# Autodesk Inventor assembly: PIVOT
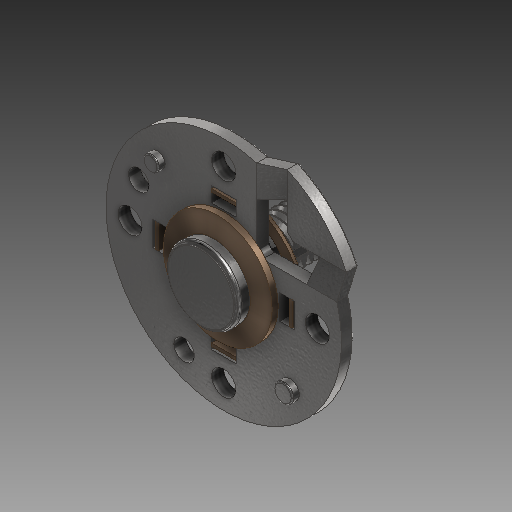
[picture p0: Inventor's stored thumbnail of the model, 512x512]
Saved by Autodesk Inventor 2017 SP1 (Build 210196100, 196)
## iProperties
Created: 2021-01-06
Part Number: PIVOT
Document SubType Name: Assembly
Designer: Napoleon
Author: Napoleon
## Documents named in this file (5)
- D:\PRYWATNE\PROJEKTY\POKÓJ\URZĄDZENIA PERYFERYJNE\DELL 1909Wf\BLOKADA.iam
- D:\PRYWATNE\PROJEKTY\POKÓJ\URZĄDZENIA PERYFERYJNE\DELL 1909Wf\ŚRUBA M8 Z WIĘCIAMI.ipt
- D:\PRYWATNE\PROJEKTY\POKÓJ\URZĄDZENIA PERYFERYJNE\DELL 1909Wf\PODKŁADKA SPRĘŻYNOWA M8X18.ipt
- D:\PRYWATNE\PROJEKTY\POKÓJ\URZĄDZENIA PERYFERYJNE\DELL 1909Wf\SŁONECZKO BLOKADY.ipt
- D:\PRYWATNE\PROJEKTY\POKÓJ\URZĄDZENIA PERYFERYJNE\DELL 1909Wf\BLOKADA PIVOT.ipt
## Components (4 placed, 4 different names)
1. ŚRUBA M8 Z WIĘCIAMI:1 — Obrotowe:1, Zestawiający:4, Zestawiający:5
2. PODKŁADKA SPRĘŻYNOWA M8X18:1 — Obrotowe:1, Zestawiający:6
3. BLOKADA PIVOT:1 — Zestawiający:4, Zestawiający:5, Zestawiający:6, Zestawiający:7
4. SŁONECZKO BLOKADY:1 — Zestawiający:7
## Relationships (5: Mate 4, RevoluteJoint 1)
- Obrotowe:1 [RevoluteJoint]: ŚRUBA M8 Z WIĘCIAMI:1 ↔ PODKŁADKA SPRĘŻYNOWA M8X18:1
- Zestawiający:4 [Mate]: ŚRUBA M8 Z WIĘCIAMI:1 ↔ BLOKADA PIVOT:1
- Zestawiający:5 [Mate]: ŚRUBA M8 Z WIĘCIAMI:1 ↔ BLOKADA PIVOT:1
- Zestawiający:6 [Mate]: PODKŁADKA SPRĘŻYNOWA M8X18:1 ↔ BLOKADA PIVOT:1
- Zestawiający:7 [Mate]: BLOKADA PIVOT:1 ↔ SŁONECZKO BLOKADY:1
